# Autodesk Inventor assembly: BD Gearbox and Bracket Assy 2
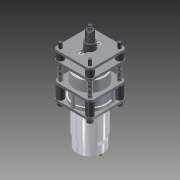
[picture p0: Inventor's stored thumbnail of the model, 180x180]
Saved by Autodesk Inventor 2012 (Build 160160000, 160)
## iProperties
Created: 2012-07-05
Part Number: BD Gearbox and Bracket Assy 2
Document SubType Name: Assembly
Designer: Bruce
Author: Bruce
## Documents named in this file (11)
- C:\Users\Bryce\Dropbox\Inventor Design Project Files\Independent Swerves\Imported Components\BD Gearbox and Bracket Assy 3.iam
- C:\Users\Bryce\Dropbox\Inventor Design Project Files\Independent Swerves\Imported Components\BD Drill motor assembly.iam
- C:\Users\Bryce\Dropbox\Inventor Design Project Files\Independent Swerves\Imported Components\BD gearbox mount block motor ring.ipt
- C:\Users\Bryce\Dropbox\Inventor Design Project Files\Independent Swerves\Imported Components\BD gearbox mount center ring.ipt
- C:\Users\Bryce\Dropbox\Inventor Design Project Files\Independent Swerves\Imported Components\Spacers BD gearbox back to ctr.ipt
- C:\Users\Bryce\Dropbox\Inventor Design Project Files\Independent Swerves\Imported Components\BD Gearbox Mount Spring plate.ipt
- C:\Users\Bryce\Dropbox\Inventor Design Project Files\Independent Swerves\Imported Components\Bolt 8-32 gearbox mount TL.ipt
- C:\Users\Bryce\Dropbox\Inventor Design Project Files\Independent Swerves\Imported Components\BD Gearbox Mount TL Spacer plate.ipt
- C:\Users\Bryce\Dropbox\Inventor Design Project Files\Independent Swerves\Imported Components\Spring BD drill motor.ipt
- C:\Users\Bryce\Dropbox\Inventor Design Project Files\Independent Swerves\Imported Components\Spacers BD Gearbox Torque Limit.ipt
- C:\Users\Bryce\Dropbox\Inventor Design Project Files\Independent Swerves\Imported Components\BD TL Plate Corner Spring.ipt
## Components (22 placed, 10 different names)
1. BD gearbox mount block motor ring:1 — Mate:5, Mate:7, Mate:8, Insert:1, Insert:2, Insert:3, Mate:12, Mate:15, Mate:17, Mate:19, Mate:22, Mate:23
2. BD Drill motor assembly:1 [sub-assembly] — Mate:5, Mate:22, Mate:23, Mate:26, Mate:27
3. Bolt 8-32 gearbox mount TL:1 — Mate:7, Mate:8, Mate:9, Mate:14, Mate:28, Mate:37
4. Bolt 8-32 gearbox mount TL:2 — Insert:3, Mate:11, Mate:21, Mate:31, Mate:39
5. Bolt 8-32 gearbox mount TL:3 — Insert:2, Mate:16, Mate:20, Mate:25, Mate:30, Mate:40
6. Bolt 8-32 gearbox mount TL:4 — Insert:1, Mate:10, Mate:18, Mate:24, Mate:29, Mate:41
7. BD gearbox mount center ring:1 — Mate:9, Mate:10, Mate:13, Mate:38, Mate:42, Mate:43, Mate:44
8. Spacers BD gearbox back to ctr:1 — Mate:11, Mate:12, Mate:13
9. Spacers BD gearbox back to ctr:2 — Mate:14, Mate:15
10. Spacers BD gearbox back to ctr:3 — Mate:16, Mate:17
11. Spacers BD gearbox back to ctr:4 — Mate:18, Mate:19
12. BD Gearbox Mount Spring plate:1 — Mate:20, Mate:21, Mate:36, Mate:45
13. BD Gearbox Mount TL Spacer plate:1 — Mate:24, Mate:25, Mate:26, Mate:32, Mate:33, Mate:34, Mate:35
14. Spring BD drill motor:1 — Mate:27, Mate:45
15. Spacers BD Gearbox Torque Limit:1 — Mate:29, Mate:32
16. Spacers BD Gearbox Torque Limit:2 — Mate:28, Mate:33
17. Spacers BD Gearbox Torque Limit:3 — Mate:30, Mate:34, Mate:36
18. Spacers BD Gearbox Torque Limit:4 — Mate:31, Mate:35
19. BD TL Plate Corner Spring:1 — Mate:37, Mate:38
20. BD TL Plate Corner Spring:2 — Mate:41, Mate:43
21. BD TL Plate Corner Spring:3 — Mate:39, Mate:44
22. BD TL Plate Corner Spring:4 — Mate:40, Mate:42
## Relationships (43: Mate 40, Insert 3)
- Mate:5: BD gearbox mount block motor ring:1 ↔ BD Drill motor assembly:1
- Mate:7: BD gearbox mount block motor ring:1 ↔ Bolt 8-32 gearbox mount TL:1
- Mate:8: BD gearbox mount block motor ring:1 ↔ Bolt 8-32 gearbox mount TL:1
- Insert:1: BD gearbox mount block motor ring:1 ↔ Bolt 8-32 gearbox mount TL:4
- Insert:2: BD gearbox mount block motor ring:1 ↔ Bolt 8-32 gearbox mount TL:3
- Insert:3: BD gearbox mount block motor ring:1 ↔ Bolt 8-32 gearbox mount TL:2
- Mate:9: Bolt 8-32 gearbox mount TL:1 ↔ BD gearbox mount center ring:1
- Mate:10: Bolt 8-32 gearbox mount TL:4 ↔ BD gearbox mount center ring:1
- Mate:11: Bolt 8-32 gearbox mount TL:2 ↔ Spacers BD gearbox back to ctr:1
- Mate:12: BD gearbox mount block motor ring:1 ↔ Spacers BD gearbox back to ctr:1
- Mate:13: BD gearbox mount center ring:1 ↔ Spacers BD gearbox back to ctr:1
- Mate:14: Bolt 8-32 gearbox mount TL:1 ↔ Spacers BD gearbox back to ctr:2
- Mate:15: BD gearbox mount block motor ring:1 ↔ Spacers BD gearbox back to ctr:2
- Mate:16: Bolt 8-32 gearbox mount TL:3 ↔ Spacers BD gearbox back to ctr:3
- Mate:17: BD gearbox mount block motor ring:1 ↔ Spacers BD gearbox back to ctr:3
- Mate:18: Bolt 8-32 gearbox mount TL:4 ↔ Spacers BD gearbox back to ctr:4
- Mate:19: BD gearbox mount block motor ring:1 ↔ Spacers BD gearbox back to ctr:4
- Mate:20: Bolt 8-32 gearbox mount TL:3 ↔ BD Gearbox Mount Spring plate:1
- Mate:21: Bolt 8-32 gearbox mount TL:2 ↔ BD Gearbox Mount Spring plate:1
- Mate:22: BD gearbox mount block motor ring:1 ↔ BD Drill motor assembly:1
- Mate:23: BD gearbox mount block motor ring:1 ↔ BD Drill motor assembly:1
- Mate:24: Bolt 8-32 gearbox mount TL:4 ↔ BD Gearbox Mount TL Spacer plate:1
- Mate:25: Bolt 8-32 gearbox mount TL:3 ↔ BD Gearbox Mount TL Spacer plate:1
- Mate:26: BD Drill motor assembly:1 ↔ BD Gearbox Mount TL Spacer plate:1
- Mate:27: BD Drill motor assembly:1 ↔ Spring BD drill motor:1
- Mate:28: Bolt 8-32 gearbox mount TL:1 ↔ Spacers BD Gearbox Torque Limit:2
- Mate:29: Bolt 8-32 gearbox mount TL:4 ↔ Spacers BD Gearbox Torque Limit:1
- Mate:30: Bolt 8-32 gearbox mount TL:3 ↔ Spacers BD Gearbox Torque Limit:3
- Mate:31: Bolt 8-32 gearbox mount TL:2 ↔ Spacers BD Gearbox Torque Limit:4
- Mate:32: BD Gearbox Mount TL Spacer plate:1 ↔ Spacers BD Gearbox Torque Limit:1
- Mate:33: BD Gearbox Mount TL Spacer plate:1 ↔ Spacers BD Gearbox Torque Limit:2
- Mate:34: BD Gearbox Mount TL Spacer plate:1 ↔ Spacers BD Gearbox Torque Limit:3
- Mate:35: BD Gearbox Mount TL Spacer plate:1 ↔ Spacers BD Gearbox Torque Limit:4
- Mate:36: BD Gearbox Mount Spring plate:1 ↔ Spacers BD Gearbox Torque Limit:3
- Mate:37: Bolt 8-32 gearbox mount TL:1 ↔ BD TL Plate Corner Spring:1
- Mate:38: BD gearbox mount center ring:1 ↔ BD TL Plate Corner Spring:1
- Mate:39: Bolt 8-32 gearbox mount TL:2 ↔ BD TL Plate Corner Spring:3
- Mate:40: Bolt 8-32 gearbox mount TL:3 ↔ BD TL Plate Corner Spring:4
- Mate:41: Bolt 8-32 gearbox mount TL:4 ↔ BD TL Plate Corner Spring:2
- Mate:42: BD gearbox mount center ring:1 ↔ BD TL Plate Corner Spring:4
- Mate:43: BD gearbox mount center ring:1 ↔ BD TL Plate Corner Spring:2
- Mate:44: BD gearbox mount center ring:1 ↔ BD TL Plate Corner Spring:3
- Mate:45: BD Gearbox Mount Spring plate:1 ↔ Spring BD drill motor:1
